# Autodesk Inventor assembly: F767ZI_MB_V1.2 1
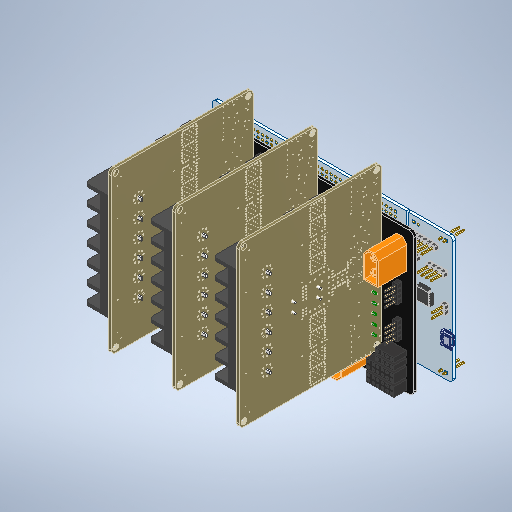
[picture p0: Inventor's stored thumbnail of the model, 512x512]
Saved by Autodesk Inventor 2025 (Build 290162010, 162A)
## iProperties
Company: Kicad
Created: 2025-02-17
Part Number: F767ZI_MB_V1.2 1
Description: KiCad electronic assembly
Document SubType Name: Assembly
Designer: tashi
Authority: Unknown
Title: F767ZI_MB_V1.2.step
Author: Pcbnew
Sending System: KiCad to STEP converter
Preprocessor: Open CASCADE STEP processor 7.8
## Documents named in this file (17)
- C:\Users\tashi\OneDrive - 学校法人立命館\Kicad\F767ZI_MB_V1.2\F767ZI_MB_V1.2\F767ZI_MB_V1.2.iam
- C:\Users\tashi\OneDrive - 学校法人立命館\Kicad\F767ZI_MB_V1.2\F767ZI_MB_V1.2\PinHeader_1x03_P2.54mm_Vertical.iam
- C:\Users\tashi\OneDrive - 学校法人立命館\Kicad\F767ZI_MB_V1.2\F767ZI_MB_V1.2\R_Axial_DIN0207_L6.3mm_D2.5mm_P10.16mm_Horizontal.iam
- C:\Users\tashi\OneDrive - 学校法人立命館\Kicad\F767ZI_MB_V1.2\F767ZI_MB_V1.2\TO-92_STM.iam
- C:\Users\tashi\OneDrive - 学校法人立命館\Kicad\F767ZI_MB_V1.2\F767ZI_MB_V1.2\PinHeader_1x04_P2.54mm_Vertical.iam
- C:\Users\tashi\OneDrive - 学校法人立命館\Kicad\F767ZI_MB_V1.2\F767ZI_MB_V1.2\PinHeader_1x02_P2.54mm_Vertical.iam
- C:\Users\tashi\OneDrive - 学校法人立命館\Kicad\F767ZI_MB_V1.2\F767ZI_MB_V1.2\PinHeader_1x11_P2.54mm_Vertical.iam
- C:\Users\tashi\OneDrive - 学校法人立命館\Kicad\F767ZI_MB_V1.2\F767ZI_MB_V1.2\PinSocket_1x04_P2.54mm_Vertical.iam
- C:\Users\tashi\OneDrive - 学校法人立命館\Kicad\F767ZI_MB_V1.2\F767ZI_MB_V1.2\XT60-M.iam
- C:\Users\tashi\OneDrive - 学校法人立命館\Kicad\F767ZI_MB_V1.2\F767ZI_MB_V1.2\PinSocket_2x06_P2.54mm_Vertical.iam
- C:\Users\tashi\OneDrive - 学校法人立命館\Kicad\F767ZI_MB_V1.2\F767ZI_MB_V1.2\PinHeader_2x10_P2.54mm_Vertical.iam
- C:\Users\tashi\OneDrive - 学校法人立命館\Kicad\F767ZI_MB_V1.2\F767ZI_MB_V1.2\PinHeader_2x17_P2.54mm_Vertical.iam
- C:\Users\tashi\OneDrive - 学校法人立命館\Kicad\F767ZI_MB_V1.2\F767ZI_MB_V1.2\PinHeader_2x08_P2.54mm_Vertical.iam
- C:\Users\tashi\OneDrive - 学校法人立命館\Kicad\F767ZI_MB_V1.2\F767ZI_MB_V1.2\PinHeader_2x15_P2.54mm_Vertical.iam
- C:\Users\tashi\OneDrive - 学校法人立命館\Kicad\F767ZI_MB_V1.2\F767ZI_MB_V1.2\F767ZI_MB_V1.2_PCB.ipt
- C:\Users\tashi\Desktop\MDD20A.STEP\MDD20A.STEP.iam
- C:\Users\tashi\OneDrive - 学校法人立命館\stepファイル\NUCLEO-F767ZI\NUCLEO-F767ZI.iam
## Components (64 placed, 62 different names)
1. 2 [sub-assembly]
2. 4 [sub-assembly]
3. 6 [sub-assembly]
4. 7 [sub-assembly]
5. 8 [sub-assembly]
6. 10 [sub-assembly]
7. 11 [sub-assembly]
8. 13 [sub-assembly]
9. 14 [sub-assembly]
10. 15 [sub-assembly]
11. 16 [sub-assembly]
12. 17 [sub-assembly]
13. 18 [sub-assembly]
14. 19 [sub-assembly]
15. 20 [sub-assembly]
16. 21 [sub-assembly]
17. 23 [sub-assembly]
18. 24 [sub-assembly]
19. 25 [sub-assembly]
20. 26 [sub-assembly]
21. 27 [sub-assembly]
22. 28 [sub-assembly]
23. 29 [sub-assembly]
24. 30 [sub-assembly]
25. 32 [sub-assembly]
26. 33 [sub-assembly]
27. 34 [sub-assembly]
28. 35 [sub-assembly]
29. 36 [sub-assembly]
30. 37 [sub-assembly]
31. 38 [sub-assembly]
32. 40 [sub-assembly]
33. 41 [sub-assembly]
34. 42 [sub-assembly]
35. 43 [sub-assembly]
36. 44 [sub-assembly]
37. 45 [sub-assembly]
38. 46 [sub-assembly]
39. 47 [sub-assembly]
40. 49 [sub-assembly]
41. 50 [sub-assembly]
42. 51 [sub-assembly]
43. 52 [sub-assembly]
44. 53 [sub-assembly]
45. 54 [sub-assembly]
46. 55 [sub-assembly]
47. 56 [sub-assembly]
48. 57 [sub-assembly]
49. 58 [sub-assembly]
50. 59 [sub-assembly]
51. 60 [sub-assembly]
52. 61 [sub-assembly]
53. 62 [sub-assembly]
54. 63 [sub-assembly]
55. 64 [sub-assembly]
56. 66 [sub-assembly]
57. 68 [sub-assembly]
58. 70 [sub-assembly]
59. 72 [sub-assembly]
60. 73
61. NUCLEO-F767ZI:1 [sub-assembly]
62. MDD20A.STEP:1 [sub-assembly]
63. MDD20A.STEP:2 [sub-assembly]
64. MDD20A.STEP:3 [sub-assembly]
## Component patterns: (3 elements, first: MDD20A.STEP:1)
